# Autodesk Inventor assembly: ShooterIdea2
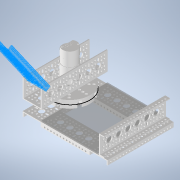
[picture p0: Inventor's stored thumbnail of the model, 180x180]
Saved by Autodesk Inventor 2021 (Build 250183000, 183)
## iProperties
Created: 2021-02-26
Part Number: ShooterIdea2
Document SubType Name: Assembly
Designer: deli
Sending System: Autodesk Inventor 2021
Preprocessor: ST-DEVELOPER v18.1
Title: C:\Users\gfellows\Downloads\ShooterIdea2.stp
Author: gfellows
## Documents named in this file (15)
- C:\Users\deli\OneDrive - Eastside Preparatory School\FTC\Ultamite Goal\ShooterIdea2.iam
- C:\Users\deli\OneDrive - Eastside Preparatory School\FTC\Ultamite Goal\5000-0002-4008.ipt
- C:\Users\deli\OneDrive - Eastside Preparatory School\FTC\Ultamite Goal\1311-0016-4008 assembly.ipt
- C:\Users\deli\OneDrive - Eastside Preparatory School\FTC\Ultamite Goal\1611-0514-4008.ipt
- C:\Users\deli\OneDrive - Eastside Preparatory School\FTC\Ultamite Goal\1613-0516-0008 assembly with 16mm OD washers.ipt
- C:\Users\deli\OneDrive - Eastside Preparatory School\FTC\Ultamite Goal\1121-0006-0168.ipt
- C:\Users\deli\OneDrive - Eastside Preparatory School\FTC\Ultamite Goal\2802-0004-0008.ipt
- C:\Users\deli\OneDrive - Eastside Preparatory School\FTC\Ultamite Goal\90657A113_ZINC-PLATED STEEL NARROW CHEESE HEAD SLOTTED SCREW.ipt
- C:\Users\deli\OneDrive - Eastside Preparatory School\FTC\Ultamite Goal\1121-0004-0120.ipt
- C:\Users\deli\OneDrive - Eastside Preparatory School\FTC\Ultamite Goal\bottom plate.ipt
- C:\Users\deli\OneDrive - Eastside Preparatory School\FTC\Ultamite Goal\1205-0001-0003.ipt
- C:\Users\deli\OneDrive - Eastside Preparatory School\FTC\Ultamite Goal\1205-0001-0003_MIR.ipt
- C:\Users\deli\OneDrive - Eastside Preparatory School\FTC\Ultamite Goal\wheel.ipt
- C:\Users\deli\OneDrive - Eastside Preparatory School\FTC\Ultamite Goal\ShooterWheel.ipt
- C:\Users\deli\OneDrive - Eastside Preparatory School\FTC\Ultamite Goal\1120-0006-0168.ipt
## Components (25 placed, 14 different names)
1. 5000-0002-4008:1 — Mate:4, Mate:8
2. 1311-0016-4008 assembly:1
3. 1611-0514-4008:1
4. 1613-0516-0008 assembly with 16mm OD washers:1
5. 1121-0006-0168:1 — Flush:1, Flush:2, Mate:9, Mate:10
6. 2802-0004-0008:1
7. 2802-0004-0008:6
8. 2802-0004-0008:7
9. 2802-0004-0008:8
10. 90657A113_ZINC-PLATED STEEL NARROW CHEESE HEAD SLOTTED SCREW:1
11. 90657A113_ZINC-PLATED STEEL NARROW CHEESE HEAD SLOTTED SCREW:2
12. 90657A113_ZINC-PLATED STEEL NARROW CHEESE HEAD SLOTTED SCREW:3
13. 90657A113_ZINC-PLATED STEEL NARROW CHEESE HEAD SLOTTED SCREW:4
14. 1121-0006-0168:3
15. 1121-0004-0120:1
16. 1121-0004-0120:2
17. bottom plate:1
18. 1205-0001-0003:1
19. 1205-0001-0003:2
20. 1205-0001-0003_MIR:1
21. 1205-0001-0003_MIR:2
22. 1121-0006-0168:4
23. wheel:2
24. ShooterWheel:1 — Mate:4, Mate:10
25. 1120-0006-0168:1 — Mate:8, Flush:1, Flush:2, Mate:9
## Relationships (6: Mate 4, Flush 2)
- Mate:4: 5000-0002-4008:1 ↔ ShooterWheel:1
- Mate:8: 5000-0002-4008:1 ↔ 1120-0006-0168:1
- Flush:1: 1121-0006-0168:1 ↔ 1120-0006-0168:1
- Flush:2: 1121-0006-0168:1 ↔ 1120-0006-0168:1
- Mate:9 (27 mm): 1121-0006-0168:1 ↔ 1120-0006-0168:1
- Mate:10: 1121-0006-0168:1 ↔ ShooterWheel:1
